# Autodesk Inventor assembly: zespoluchwyt
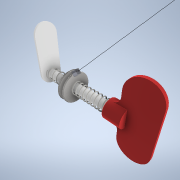
[picture p0: Inventor's stored thumbnail of the model, 180x180]
Saved by Autodesk Inventor 2021 (Build 250183000, 183)
## iProperties
Created: 2021-06-22
Part Number: zespoluchwyt
Document SubType Name: Assembly
Designer: Wojciech Wołczek
Author: Wojciech Wołczek
## Documents named in this file (6)
- D:\OneDrive\Documents\autodesk\uchwytokno\zespoluchwyt.iam
- D:\OneDrive\Documents\autodesk\uchwytokno\uchwyt1.ipt
- D:\OneDrive\Documents\autodesk\uchwytokno\podkl.ipt
- D:\OneDrive\Documents\autodesk\uchwytokno\sprezy23.ipt
- D:\OneDrive\Documents\autodesk\uchwytokno\sprezy2.ipt
- D:\OneDrive\Documents\autodesk\uchwytokno\raczka.ipt
## Components (6 placed, 5 different names)
1. uchwyt1:1 — Równoległe:1, Równoległe:3, Zestawiające:1
2. podkl:1 — Równoległe:4, Równoległe:5, Zestawiające:5
3. sprezy23:1 — Równoległe:6
4. podkl:2 — Zestawiające:4, Zestawiające:5, Zestawiające:6
5. sprezy2:1 — Równoległe:8
6. raczka:1 — Równoległe:9
## Relationships (14: Flush 8, Mate 6)
- Równoległe:1 [Flush]: uchwyt1:1
- Równoległe:3 [Flush] (20 mm): uchwyt1:1
- Równoległe:4 [Flush]: podkl:1
- Równoległe:5 [Flush]: podkl:1
- Zestawiające:1 [Mate]: uchwyt1:1
- Zestawiające:2 [Mate]
- Zestawiające:3 [Mate]
- Równoległe:6 [Flush]: sprezy23:1
- Zestawiające:4 [Mate]: podkl:2
- Zestawiające:5 [Mate] (3 mm): podkl:1 ↔ podkl:2
- Zestawiające:6 [Mate]: podkl:2
- Równoległe:7 [Flush] (-60 mm)
- Równoległe:8 [Flush]: sprezy2:1
- Równoległe:9 [Flush]: raczka:1
